# Autodesk Inventor assembly: Complete Drone Assembly
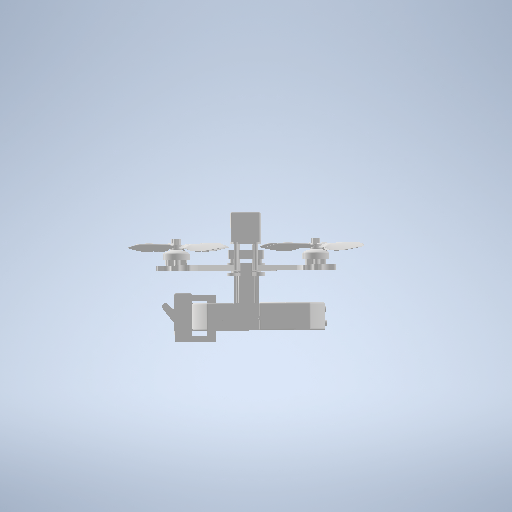
[picture p0: Inventor's stored thumbnail of the model, 512x512]
Saved by Autodesk Inventor 2025 (Build 290162010, 162A)
## iProperties
Created: 2024-06-19
Part Number: Complete Drone Assembly
Document SubType Name: Assembly
Designer: ppatel269
Author: ppatel269
## Documents named in this file (14)
- D:\All Drone Parts\Complete Drone Assembly.iam
- D:\All Drone Parts\Drone Parts.ipt\Drone Frame.ipt
- D:\All Drone Parts\Drone Parts.ipt\Drone Droppin Mech.ipt
- D:\All Drone Parts\Drone Parts.ipt\Drone Prop.ipt
- D:\All Drone Parts\rod.ipt
- D:\All Drone Parts\Drone Parts.ipt\Drone Droppin Mech Right.ipt
- D:\All Drone Parts\Drone Parts.ipt\Droppin Mech Clamp.ipt
- D:\All Drone Parts\Drone Parts.ipt\Rod Cap.ipt
- D:\All Drone Parts\Drone Parts.ipt\Drone Droppin Mech Left.ipt
- D:\All Drone Parts\Drone Parts.ipt\Camera Mount.ipt
- D:\All Drone Parts\Drone Parts.ipt\Laser Mount.ipt
- D:\All Drone Parts\Drone Parts.ipt\Servo Attatchment.ipt
- D:\All Drone Parts\Servo.ipt
- D:\All Drone Parts\Spring.ipt
## Components (17 placed, 13 different names)
1. Drone Frame:1 — Mate:1, Mate:3, Mate:5, Mate:6, Mate:7, Mate:8, Mate:18, Mate:19, Mate:21, Flush:1, Mate:43, Mate:44
2. Drone Droppin Mech:1 — Mate:1, Mate:2, Mate:22, Mate:25, Flush:1, Mate:45, Mate:46, Mate:49, Mate:54, Flush:3, Flush:4, Mate:62
3. Drone Prop:1 — Mate:43, Mate:44
4. Drone Prop:2 — Mate:10, Mate:21
5. Drone Prop:3 — Mate:15, Mate:18
6. Drone Prop:4 — Mate:9, Mate:19
7. Drone Droppin Mech Right:1 — Mate:27, Mate:29, Mate:47, Mate:48, Mate:49, Mate:50, Mate:51, Flush:2
8. Rod Cap:1 — Mate:32, Mate:33, Mate:52, Mate:53, Mate:61, Mate:64
9. Servo Attatchment:1 — Mate:60, Flush:8, Flush:9
10. Laser Mount:1 — Mate:55, Flush:5, Mate:56
11. Servo:1 — Mate:59, Flush:6, Flush:7, Mate:60, Flush:9
12. rod:1 — Mate:46, Mate:48, Mate:58
13. rod:2 — Mate:45, Mate:47, Mate:52, Mate:53, Mate:57, Mate:63
14. Droppin Mech Clamp:1 — Mate:50, Mate:51, Flush:2, Mate:56
15. Camera Mount:1 — Mate:54, Flush:3, Flush:4, Mate:55, Flush:5
16. Drone Droppin Mech Left:1 — Mate:57, Mate:58, Mate:59, Flush:6, Flush:7, Flush:8, Mate:61, Mate:62
17. Spring:1 — Mate:63, Mate:64
## Relationships (55: Mate 46, Flush 9)
- Mate:1: Drone Frame:1 ↔ Drone Droppin Mech:1
- Mate:2: Drone Droppin Mech:1
- Mate:3: Drone Frame:1
- Mate:4
- Mate:5: Drone Frame:1
- Mate:6: Drone Frame:1
- Mate:7: Drone Frame:1
- Mate:8: Drone Frame:1
- Mate:9: Drone Prop:4
- Mate:10: Drone Prop:2
- Mate:11
- Mate:12
- Mate:15: Drone Prop:3
- Mate:16
- Mate:17
- Mate:18: Drone Frame:1 ↔ Drone Prop:3
- Mate:19: Drone Frame:1 ↔ Drone Prop:4
- Mate:21: Drone Frame:1 ↔ Drone Prop:2
- Mate:22: Drone Droppin Mech:1
- Mate:25: Drone Droppin Mech:1
- Flush:1: Drone Frame:1 ↔ Drone Droppin Mech:1
- Mate:27: Drone Droppin Mech Right:1
- Mate:29: Drone Droppin Mech Right:1
- Mate:32: Rod Cap:1
- Mate:33: Rod Cap:1
- Mate:43: Drone Frame:1 ↔ Drone Prop:1
- Mate:44: Drone Frame:1 ↔ Drone Prop:1
- Mate:45: Drone Droppin Mech:1 ↔ rod:2
- Mate:46: Drone Droppin Mech:1 ↔ rod:1
- Mate:47: Drone Droppin Mech Right:1 ↔ rod:2
- Mate:48: Drone Droppin Mech Right:1 ↔ rod:1
- Mate:49: Drone Droppin Mech:1 ↔ Drone Droppin Mech Right:1
- Mate:50: Drone Droppin Mech Right:1 ↔ Droppin Mech Clamp:1
- Mate:51: Drone Droppin Mech Right:1 ↔ Droppin Mech Clamp:1
- Flush:2: Drone Droppin Mech Right:1 ↔ Droppin Mech Clamp:1
- Mate:52: Rod Cap:1 ↔ rod:2
- Mate:53: Rod Cap:1 ↔ rod:2
- Mate:54: Drone Droppin Mech:1 ↔ Camera Mount:1
- Flush:3: Drone Droppin Mech:1 ↔ Camera Mount:1
- Flush:4: Drone Droppin Mech:1 ↔ Camera Mount:1
- Mate:55: Laser Mount:1 ↔ Camera Mount:1
- Flush:5: Laser Mount:1 ↔ Camera Mount:1
- Mate:56: Laser Mount:1 ↔ Droppin Mech Clamp:1
- Mate:57: rod:2 ↔ Drone Droppin Mech Left:1
- Mate:58: rod:1 ↔ Drone Droppin Mech Left:1
- Mate:59: Servo:1 ↔ Drone Droppin Mech Left:1
- Flush:6: Servo:1 ↔ Drone Droppin Mech Left:1
- Flush:7: Servo:1 ↔ Drone Droppin Mech Left:1
- Mate:60: Servo Attatchment:1 ↔ Servo:1
- Flush:8: Servo Attatchment:1 ↔ Drone Droppin Mech Left:1
- Flush:9: Servo Attatchment:1 ↔ Servo:1
- Mate:61 (15 mm): Rod Cap:1 ↔ Drone Droppin Mech Left:1
- Mate:62: Drone Droppin Mech:1 ↔ Drone Droppin Mech Left:1
- Mate:63: rod:2 ↔ Spring:1
- Mate:64: Rod Cap:1 ↔ Spring:1
